# Autodesk Inventor assembly: mizuno-probe-head
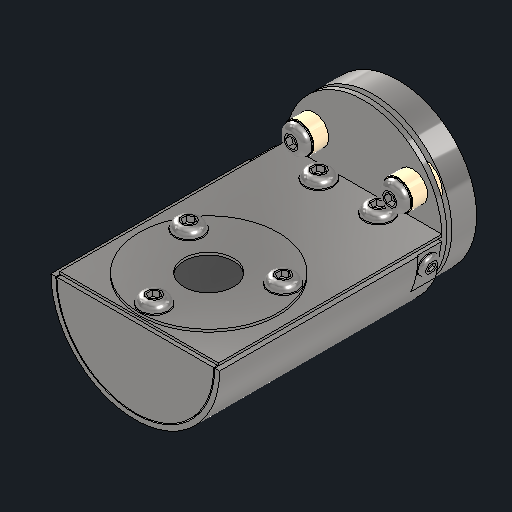
[picture p0: Inventor's stored thumbnail of the model, 512x512]
Saved by Autodesk Inventor 2027.1 (Build 311270010, 270A)
## iProperties
Created: 2026-10-08
Part Number: mizuno-probe-head
Document SubType Name: Assembly
Designer: queezz
Author: queezz
## Documents named in this file (14)
- C:\Users\queezz\Dropbox\Drawings\pihti-cad\bellows-probe\mizuno-probe-head.iam
- C:\Users\queezz\Dropbox\Drawings\pihti-cad\BoronProbe_2026\parts\B_probehead_5.ipt
- C:\Users\queezz\Dropbox\Drawings\pihti-cad\BoronProbe_2026\parts\B_holder_sub_5.ipt
- C:\Users\queezz\Dropbox\Drawings\pihti-cad\ContentCenter\Fastners\M3x6-BHCS.ipt
- C:\Users\queezz\Dropbox\Drawings\pihti-cad\ContentCenter\Ceramics\ceramic_bushing_M3-v1.ipt
- C:\Users\queezz\Dropbox\Drawings\pihti-cad\ContentCenter\Ceramics\ceramic_washer_M4_v1.ipt
- C:\Users\queezz\Dropbox\Drawings\pihti-cad\BoronProbe_2026\parts\B_pipe_cylinder_5.ipt
- C:\Users\queezz\Dropbox\Drawings\pihti-cad\BoronProbe_2026\parts\B_shield_5.iam
- C:\Users\queezz\Dropbox\Drawings\pihti-cad\BoronProbe_2026\parts\ceramic_spacer_d3-13.ipt
- C:\Users\queezz\Dropbox\Drawings\pihti-cad\BoronProbe_2026\parts\ceramic_2-hole-spacer_d3-13.ipt
- C:\Users\queezz\Dropbox\Drawings\pihti-cad\BoronProbe_2026\parts\M2-4_screw.ipt
- C:\Users\queezz\Dropbox\Drawings\pihti-cad\BoronProbe_2026\parts\substrate.ipt
- C:\Users\queezz\Dropbox\Drawings\pihti-cad\ContentCenter\Fastners\M3-nut.ipt
- C:\Users\queezz\Dropbox\Drawings\pihti-cad\BoronProbe_2026\parts\B_holder_up_5.ipt
## Components (28 placed, 13 different names)
1. B_probehead_5:1
2. B_holder_sub_5:1
3. Broached Hexagon Socket Button Head Cap Screw - Metric M3 x 0.5 x 6:1
4. Broached Hexagon Socket Button Head Cap Screw - Metric M3 x 0.5 x 6:2
5. Broached Hexagon Socket Button Head Cap Screw - Metric M3 x 0.5 x 6:3
6. ceramic_bushing_M3-v1:1
7. ceramic_bushing_M3-v1:2
8. ceramic_bushing_M3-v1:3
9. ceramic_washer_M4_v1:1
10. ceramic_washer_M4_v1:2
11. ceramic_washer_M4_v1:3
12. Broached Hexagon Socket Button Head Cap Screw - Metric M3 x 0.5 x 6:4
13. Broached Hexagon Socket Button Head Cap Screw - Metric M3 x 0.5 x 6:5
14. B_pipe_cylinder_5:1
15. B_shield_5:1 [sub-assembly]
16. ceramic_spacer_d3-13:1
17. ceramic_spacer_d3-13:2
18. ceramic_2-hole-spacer_d3-13:1
19. M2-4_screw:1
20. M2-4_screw:2
21. substrate:1
22. JIS B 1181 Style 1 - Metric A M3:1
23. JIS B 1181 Style 1 - Metric A M3:2
24. JIS B 1181 Style 1 - Metric A M3:3
25. B_holder_up_5:1
26. Broached Hexagon Socket Button Head Cap Screw - Metric M3 x 0.5 x 6:6
27. Broached Hexagon Socket Button Head Cap Screw - Metric M3 x 0.5 x 6:7
28. Broached Hexagon Socket Button Head Cap Screw - Metric M3 x 0.5 x 6:8
## Relationships (58: Mate 55, Flush 3)
- [Mate]: B_probehead_5:1 ↔ B_holder_sub_5:1
- [Mate]: B_probehead_5:1 ↔ B_holder_sub_5:1
- [Mate]: B_probehead_5:1 ↔ B_holder_sub_5:1
- [Mate]: B_probehead_5:1 ↔ Broached Hexagon Socket Button Head Cap Screw - Metric M3 x 0.5 x 6:1
- [Mate]: B_holder_sub_5:1 ↔ Broached Hexagon Socket Button Head Cap Screw - Metric M3 x 0.5 x 6:1
- [Mate]: B_probehead_5:1 ↔ Broached Hexagon Socket Button Head Cap Screw - Metric M3 x 0.5 x 6:2
- [Mate]: B_holder_sub_5:1 ↔ Broached Hexagon Socket Button Head Cap Screw - Metric M3 x 0.5 x 6:2
- [Mate]: B_probehead_5:1 ↔ ceramic_bushing_M3-v1:3
- [Mate]: B_probehead_5:1 ↔ ceramic_bushing_M3-v1:3
- [Mate]: B_probehead_5:1 ↔ ceramic_bushing_M3-v1:2
- [Mate]: B_probehead_5:1 ↔ ceramic_bushing_M3-v1:2
- [Mate]: B_probehead_5:1 ↔ ceramic_bushing_M3-v1:1
- [Mate]: B_probehead_5:1 ↔ ceramic_bushing_M3-v1:1
- [Mate]: B_probehead_5:1 ↔ ceramic_washer_M4_v1:2
- [Mate]: ceramic_bushing_M3-v1:2 ↔ ceramic_washer_M4_v1:2
- [Mate]: B_probehead_5:1 ↔ ceramic_washer_M4_v1:1
- [Mate]: ceramic_bushing_M3-v1:3 ↔ ceramic_washer_M4_v1:1
- [Mate]: B_probehead_5:1 ↔ ceramic_washer_M4_v1:3
- [Mate]: ceramic_bushing_M3-v1:1 ↔ ceramic_washer_M4_v1:3
- [Mate]: ceramic_bushing_M3-v1:1 ↔ Broached Hexagon Socket Button Head Cap Screw - Metric M3 x 0.5 x 6:5
- [Mate]: ceramic_bushing_M3-v1:1 ↔ Broached Hexagon Socket Button Head Cap Screw - Metric M3 x 0.5 x 6:5
- [Mate]: ceramic_bushing_M3-v1:3 ↔ Broached Hexagon Socket Button Head Cap Screw - Metric M3 x 0.5 x 6:4
- [Mate]: ceramic_bushing_M3-v1:3 ↔ Broached Hexagon Socket Button Head Cap Screw - Metric M3 x 0.5 x 6:4
- [Mate]: Broached Hexagon Socket Button Head Cap Screw - Metric M3 x 0.5 x 6:3 ↔ ceramic_bushing_M3-v1:2
- [Mate]: Broached Hexagon Socket Button Head Cap Screw - Metric M3 x 0.5 x 6:3 ↔ ceramic_bushing_M3-v1:2
- [Mate]: ceramic_washer_M4_v1:2 ↔ B_pipe_cylinder_5:1
- [Mate]: ceramic_washer_M4_v1:1 ↔ B_pipe_cylinder_5:1
- [Mate]: ceramic_washer_M4_v1:3 ↔ B_pipe_cylinder_5:1
- [Mate]: B_probehead_5:1 ↔ B_shield_5:1
- [Mate]: B_probehead_5:1 ↔ B_shield_5:1
- [Mate]: B_probehead_5:1 ↔ B_shield_5:1
- [Mate]: B_probehead_5:1 ↔ ceramic_spacer_d3-13:1
- [Flush]: B_probehead_5:1 ↔ ceramic_spacer_d3-13:1
- [Mate]: B_probehead_5:1 ↔ ceramic_spacer_d3-13:2
- [Flush]: B_probehead_5:1 ↔ ceramic_spacer_d3-13:2
- [Mate]: B_probehead_5:1 ↔ ceramic_2-hole-spacer_d3-13:1
- [Flush]: B_probehead_5:1 ↔ ceramic_2-hole-spacer_d3-13:1
- [Mate]: B_shield_5:1 ↔ M2-4_screw:1
- [Mate]: B_shield_5:1 ↔ M2-4_screw:1
- [Mate]: B_shield_5:1 ↔ M2-4_screw:2
- [Mate]: B_shield_5:1 ↔ M2-4_screw:2
- [Mate]: B_holder_sub_5:1 ↔ substrate:1
- [Mate]: B_holder_sub_5:1 ↔ substrate:1
- [Mate]: B_holder_sub_5:1 ↔ JIS B 1181 Style 1 - Metric A M3:1
- [Mate]: B_holder_sub_5:1 ↔ JIS B 1181 Style 1 - Metric A M3:1
- [Mate]: B_holder_sub_5:1 ↔ JIS B 1181 Style 1 - Metric A M3:3
- [Mate]: B_holder_sub_5:1 ↔ JIS B 1181 Style 1 - Metric A M3:3
- [Mate]: B_holder_sub_5:1 ↔ JIS B 1181 Style 1 - Metric A M3:2
- [Mate]: B_holder_sub_5:1 ↔ JIS B 1181 Style 1 - Metric A M3:2
- [Mate]: substrate:1 ↔ B_holder_up_5:1
- [Mate]: JIS B 1181 Style 1 - Metric A M3:3 ↔ B_holder_up_5:1
- [Mate]: B_holder_sub_5:1 ↔ B_holder_up_5:1
- [Mate]: B_holder_up_5:1 ↔ Broached Hexagon Socket Button Head Cap Screw - Metric M3 x 0.5 x 6:6
- [Mate]: B_holder_up_5:1 ↔ Broached Hexagon Socket Button Head Cap Screw - Metric M3 x 0.5 x 6:6
- [Mate]: B_holder_up_5:1 ↔ Broached Hexagon Socket Button Head Cap Screw - Metric M3 x 0.5 x 6:7
- [Mate]: B_holder_up_5:1 ↔ Broached Hexagon Socket Button Head Cap Screw - Metric M3 x 0.5 x 6:7
- [Mate]: B_holder_up_5:1 ↔ Broached Hexagon Socket Button Head Cap Screw - Metric M3 x 0.5 x 6:8
- [Mate]: B_holder_up_5:1 ↔ Broached Hexagon Socket Button Head Cap Screw - Metric M3 x 0.5 x 6:8
## Named parameters: d38_d41 = 0 mm, d39_d42 = 0 mm, d40_d43 = 0 mm, d41_d44 = 0 mm, d42_d45 = 0 mm, d43_d46 = 0 mm, d44_d49 = 0 mm, d45_d50 = 0 mm, d46_d51 = 0 mm, d47_d56 = 0 mm, d48_d57 = 0 mm
